# Autodesk Inventor assembly: MSK01-05A
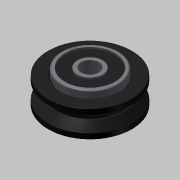
[picture p0: Inventor's stored thumbnail of the model, 180x180]
Saved by Autodesk Inventor 2013 (Build 170138000, 138)
## iProperties
Created: 2012-01-16
Part Number: MSK01-05A
Document SubType Name: Assembly
Designer: ERF
Description: Dual Bearing V Wheel Kit
Stock Number: MSK01-05A
Author: ERF
Title: v-wheel assembly
## Documents named in this file (4)
- C:\Users\Brett\Documents\Autodesk\Projects\Shapeoko_v1i\Assemblies\MSK01-05A.iam
- C:\Users\Brett\Documents\Autodesk\Projects\Shapeoko_v1i\Parts\B17021.ipt
- C:\Users\Brett\Documents\Autodesk\Projects\Shapeoko_v1i\Parts\BEARING_5_16_5.ipt
- C:\Users\Brett\Documents\Autodesk\Projects\Shapeoko_v1i\Parts\B18026.ipt
## Components (4 placed, 3 different names)
1. B17021:1 — Insert:1, Insert:3
2. BEARING_5_16_5:1 — Insert:3, Insert:4
3. B18026:1 — Insert:4
4. BEARING_5_16_5:2 — Insert:1
## Relationships (3: Insert 3)
- Insert:1: B17021:1 ↔ BEARING_5_16_5:2
- Insert:3: B17021:1 ↔ BEARING_5_16_5:1
- Insert:4: BEARING_5_16_5:1 ↔ B18026:1
